# Autodesk Inventor assembly: Holotape
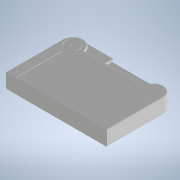
[picture p0: Inventor's stored thumbnail of the model, 180x180]
Saved by Autodesk Inventor 2021 (Build 250183000, 183)
## iProperties
Created: 2021-05-07
Part Number: Holotape
Document SubType Name: Assembly
Designer: trent
Author: trent
## Documents named in this file (3)
- C:\Users\trent\OneDrive - wmpenn.edu\Personal\PIP-Boy 6400 Mk.I\Holotape.iam
- C:\Users\trent\OneDrive - wmpenn.edu\Personal\PIP-Boy 6400 Mk.I\PIP-Boy Extras_HolotapeBottomHalf.ipt
- C:\Users\trent\OneDrive - wmpenn.edu\Personal\PIP-Boy 6400 Mk.I\PIP-Boy Extras_HolotapeTopHalf.ipt
## Components (2 placed, 2 different names)
1. PIP-Boy Extras_HolotapeBottomHalf:1 — Mate:1, Flush:1, Flush:2
2. PIP-Boy Extras_HolotapeTopHalf:1 — Mate:1, Flush:1, Flush:2
## Relationships (3: Flush 2, Mate 1)
- Mate:1: PIP-Boy Extras_HolotapeBottomHalf:1 ↔ PIP-Boy Extras_HolotapeTopHalf:1
- Flush:1: PIP-Boy Extras_HolotapeBottomHalf:1 ↔ PIP-Boy Extras_HolotapeTopHalf:1
- Flush:2: PIP-Boy Extras_HolotapeBottomHalf:1 ↔ PIP-Boy Extras_HolotapeTopHalf:1
